# Autodesk Inventor assembly: TwoSparkMaxPlate
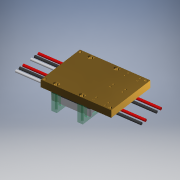
[picture p0: Inventor's stored thumbnail of the model, 180x180]
Saved by Autodesk Inventor 2019 (Build 230136000, 136)
## iProperties
Created: 2019-12-12
Part Number: TwoSparkMaxPlate
Document SubType Name: Assembly
Designer: james
Author: james
## Documents named in this file (4)
- F:\JimsRobot\FIRSTRobots\Design\Library\Jims\TwoSparkMaxPlate.iam
- F:\JimsRobot\FIRSTRobots\Design\Library\RevRobotics\REV-11-2158.ipt
- F:\JimsRobot\FIRSTRobots\Design\Library\Jims\SparkMaxPlate.ipt
- F:\JimsRobot\FIRSTRobots\Design\Library\Jims\SparkMaxTop.ipt
## Components (5 placed, 3 different names)
1. REV-11-2158:1 — Mate:1, Mate:3, Flush:1
2. REV-11-2158:2 — Mate:2, Mate:3
3. SparkMaxPlate:1 — Mate:1, Mate:2, Mate:4, Mate:5, Mate:6, Mate:7, Mate:8, Mate:9, Flush:1
4. SparkMaxTop:1 — Mate:5, Mate:6, Mate:7
5. SparkMaxTop:2 — Mate:4, Mate:8, Mate:9
## Relationships (10: Mate 9, Flush 1)
- Mate:1: REV-11-2158:1 ↔ SparkMaxPlate:1
- Mate:2: REV-11-2158:2 ↔ SparkMaxPlate:1
- Mate:3: REV-11-2158:1 ↔ REV-11-2158:2
- Mate:4: SparkMaxPlate:1 ↔ SparkMaxTop:2
- Mate:5: SparkMaxPlate:1 ↔ SparkMaxTop:1
- Mate:6: SparkMaxPlate:1 ↔ SparkMaxTop:1
- Mate:7: SparkMaxPlate:1 ↔ SparkMaxTop:1
- Mate:8: SparkMaxPlate:1 ↔ SparkMaxTop:2
- Mate:9: SparkMaxPlate:1 ↔ SparkMaxTop:2
- Flush:1 (10.16 mm): REV-11-2158:1 ↔ SparkMaxPlate:1
